# Autodesk Inventor assembly: steering_hub_assembly_right
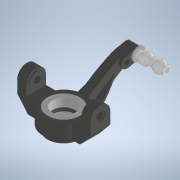
[picture p0: Inventor's stored thumbnail of the model, 180x180]
Saved by Autodesk Inventor 2020 (Build 240168000, 168)
## iProperties
Created: 2019-12-09
Part Number: steering_hub_assembly_right
Document SubType Name: Assembly
Designer: maste
Author: maste
## Documents named in this file (7)
- C:\Users\maste\Documents\GitHub\autobot\robot_model\steering_hub_assembly_right.iam
- C:\Users\maste\Documents\GitHub\autobot\robot_model\RCT-P006_steering_knuckle_right_OK.ipt
- C:\Users\maste\Documents\GitHub\autobot\robot_model\B6700ZZ.ipt
- C:\Users\maste\Documents\GitHub\autobot\robot_model\BR115ZZ.ipt
- C:\Users\maste\Documents\GitHub\autobot\robot_model\RCT-H019.ipt
- C:\Users\maste\Documents\GitHub\autobot\robot_model\RCT-H022_washer_31_60_05.ipt
- C:\Users\maste\Documents\GitHub\autobot\robot_model\H016.ipt
## Components (8 placed, 6 different names)
1. RCT-P006_steering_knuckle_right_OK:1 — Mate:1, Mate:2, Mate:3, Mate:4, Mate:5, Mate:6, Mate:7, Mate:8, Mate:9, Mate:10, Mate:12
2. B6700ZZ:1 — Mate:1, Mate:2
3. BR115ZZ:1 — Mate:3, Mate:4
4. RCT-H019:1 — Mate:5, Mate:6
5. RCT-H019:2 — Mate:7, Mate:8
6. RCT-H022_washer_31_60_05:1 — Mate:9, Mate:10, Mate:11
7. H016:1 — Mate:11, Mate:12, Mate:13, Mate:14
8. H016:2 — Mate:13, Mate:14
## Relationships (14: Mate 14)
- Mate:1: RCT-P006_steering_knuckle_right_OK:1 ↔ B6700ZZ:1
- Mate:2: RCT-P006_steering_knuckle_right_OK:1 ↔ B6700ZZ:1
- Mate:3: RCT-P006_steering_knuckle_right_OK:1 ↔ BR115ZZ:1
- Mate:4: RCT-P006_steering_knuckle_right_OK:1 ↔ BR115ZZ:1
- Mate:5: RCT-P006_steering_knuckle_right_OK:1 ↔ RCT-H019:1
- Mate:6: RCT-P006_steering_knuckle_right_OK:1 ↔ RCT-H019:1
- Mate:7: RCT-P006_steering_knuckle_right_OK:1 ↔ RCT-H019:2
- Mate:8: RCT-P006_steering_knuckle_right_OK:1 ↔ RCT-H019:2
- Mate:9: RCT-P006_steering_knuckle_right_OK:1 ↔ RCT-H022_washer_31_60_05:1
- Mate:10: RCT-P006_steering_knuckle_right_OK:1 ↔ RCT-H022_washer_31_60_05:1
- Mate:11: RCT-H022_washer_31_60_05:1 ↔ H016:1
- Mate:12: RCT-P006_steering_knuckle_right_OK:1 ↔ H016:1
- Mate:13: H016:1 ↔ H016:2
- Mate:14: H016:1 ↔ H016:2
